# Autodesk Inventor assembly: YAxis_Carriage
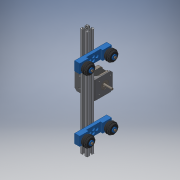
[picture p0: Inventor's stored thumbnail of the model, 180x180]
Saved by Autodesk Inventor 2019.4 (Build 234330000, 330)
## iProperties
Created: 2021-02-02
Part Number: YAxis_Carriage
Document SubType Name: Assembly
Designer: Jorian Brusind
Author: Jorian Brusind
## Documents named in this file (5)
- C:\Users\Jorian Brusind\Documents\GitHub\PersonalProjects\HyperRail\Inventor Files\YAxis_Carriage.iam
- C:\Users\Jorian Brusind\Documents\GitHub\PersonalProjects\Inventor Projects\Useful models\8020_Sets\IPT_20_Series\IPT_20_Series\20-2020_300mm.ipt
- C:\Users\Jorian Brusind\Documents\GitHub\PersonalProjects\Inventor Projects\Useful models\NEMA_Steppers\nema-17-stepper-motor-with-v2-damper-1.snapshot.3\Nema 17  Stepper Motor length 34mm.ipt
- C:\Users\Jorian Brusind\Documents\GitHub\PersonalProjects\Inventor Projects\Useful models\NEMA_Steppers\nema-17-steel-motor-mount-1.snapshot.2\NEMA17 - Steel Motor Mount.ipt
- C:\Users\Jorian Brusind\Documents\GitHub\PersonalProjects\HyperRail\Inventor Files\Roller_Bracket_40mm.iam
## Components (5 placed, 4 different names)
1. 20-2020_300mm:1 — Mate:3, Flush:1, Flush:2, Mate:9, Mate:10, Mate:11, Mate:12, Flush:3
2. Nema 17  Stepper Motor length 34mm:1 — Mate:4, Mate:5, Mate:6
3. NEMA17 - Steel Motor Mount:1 — Mate:3, Mate:4, Mate:5, Mate:6, Flush:3, Mate:13
4. Roller_Bracket_40mm:1 [sub-assembly] — Flush:2, Mate:10, Mate:11, Mate:13
5. Roller_Bracket_40mm:2 [sub-assembly] — Flush:1, Mate:9, Mate:12
## Relationships (12: Mate 9, Flush 3)
- Mate:3: 20-2020_300mm:1 ↔ NEMA17 - Steel Motor Mount:1
- Mate:4: Nema 17  Stepper Motor length 34mm:1 ↔ NEMA17 - Steel Motor Mount:1
- Mate:5: Nema 17  Stepper Motor length 34mm:1 ↔ NEMA17 - Steel Motor Mount:1
- Mate:6: Nema 17  Stepper Motor length 34mm:1 ↔ NEMA17 - Steel Motor Mount:1
- Flush:1 (50 mm): 20-2020_300mm:1 ↔ Roller_Bracket_40mm:2
- Flush:2 (50 mm): 20-2020_300mm:1 ↔ Roller_Bracket_40mm:1
- Mate:9 (10 mm): 20-2020_300mm:1 ↔ Roller_Bracket_40mm:2
- Mate:10 (10 mm): 20-2020_300mm:1 ↔ Roller_Bracket_40mm:1
- Mate:11: 20-2020_300mm:1 ↔ Roller_Bracket_40mm:1
- Mate:12: 20-2020_300mm:1 ↔ Roller_Bracket_40mm:2
- Flush:3: 20-2020_300mm:1 ↔ NEMA17 - Steel Motor Mount:1
- Mate:13 (50 mm): NEMA17 - Steel Motor Mount:1 ↔ Roller_Bracket_40mm:1
